# Autodesk Inventor assembly: Top Plate Assembly
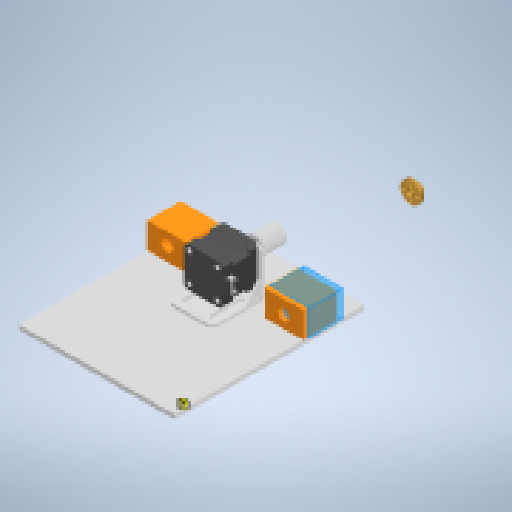
[picture p0: Inventor's stored thumbnail of the model, 512x512]
Saved by Autodesk Inventor 2023.1 (Build 271208000, 208)
## iProperties
Created: 2023-01-31
Part Number: Top Plate Assembly
Document SubType Name: Assembly
Designer: dmargari
Author: dmargari
## iProperties of the stored document Part9.ipt
Created: 2023-02-01
Part Number: Part9
Material: Generic
Document SubType Name: Modeling
Designer: dmargari
Density: 1 g/cm^3
Appearance: Default
Author: dmargari
## iProperties of the stored document JST 2.0 PH - 6 Pin v5.iam
Created: 2023-02-01
Part Number: JST 2.0 PH - 6 Pin
Document SubType Name: Assembly
Designer: dmargari
Author: dmargari
## iProperties of the stored document Shaft.ipt
Created: 2023-02-01
Part Number: Shaft
Material: Steel
Document SubType Name: Modeling
Designer: dmargari
Density: 7.85 g/cm^3
Appearance: Default
Author: dmargari
## iProperties of the stored document M3 x 15mm.iam
Created: 2023-02-01
Part Number: M3 x 15mm
Document SubType Name: Assembly
Designer: dmargari
Author: dmargari
## iProperties of the stored document Pin.ipt
Created: 2023-02-01
Part Number: Pin
Material: Gold
Document SubType Name: Modeling
Designer: dmargari
Density: 19.3 g/cm^3
Appearance: Default
Author: dmargari
## iProperties of the stored document Part13.ipt
Created: 2023-02-01
Part Number: Part13
Material: Generic
Document SubType Name: Modeling
Designer: dmargari
Density: 1 g/cm^3
Appearance: Default
Author: dmargari
## iProperties of the stored document Part11.ipt
Created: 2023-02-01
Part Number: Part11
Material: Generic
Document SubType Name: Modeling
Designer: dmargari
Density: 1 g/cm^3
Appearance: Default
Author: dmargari
## iProperties of the stored document Nema 17 40mm.iam
Created: 2020-03-04
Part Number: Nema 17 40mm
Document SubType Name: Assembly
Designer: dmargari
Sending System: Autodesk Translation Framework v8.12.0.6
Preprocessor: ST-DEVELOPER v18
Title: /Users/nikolajthranecarlsen/Library/Mobile Documents/com~apple~CloudDocs/3D programmer/Rulle gardin/Nema 17 40mm.step
## iProperties of the stored document Mid.ipt
Created: 2023-02-01
Part Number: Mid
Material: Steel
Document SubType Name: Modeling
Designer: dmargari
Density: 7.85 g/cm^3
Appearance: Default
Author: dmargari
## Documents named in this file (14)
- \\icnas3.cc.ic.ac.uk\dmargari\Inventor\Autosampler V3\Top Plate Assembly.iam
- \\icnas3.cc.ic.ac.uk\dmargari\Inventor\Autosampler V3\Top Plate.ipt
- **\\icnas3.cc.ic.ac.uk\dmargari\Inventor\Autosampler V3\Top Plate Assembly.iam*LocalDocs*xAaaaqgbaAaaaaaaaAaaaasfj3f*Nema 17 40mm.iam
- \\icnas3.cc.ic.ac.uk\dmargari\Inventor\Autosampler V3\3rd-party-models\ACME Brass Nut.ipt
- \\icnas3.cc.ic.ac.uk\dmargari\Inventor\Autosampler V3\3rd-party-models\Shaft Coupler 5mm 8mm.ipt
- **\\icnas3.cc.ic.ac.uk\dmargari\Inventor\Autosampler V3\Top Plate Assembly.iam*LocalDocs*xAaaaaubaAaaaaaaaAaaaaqnuYd*Part9.ipt
- **\\icnas3.cc.ic.ac.uk\dmargari\Inventor\Autosampler V3\Top Plate Assembly.iam*LocalDocs*xAaaaalbaAaaaaaaaAaaaq2mvYc*JST 2.0 PH - 6 Pin v5.iam
- **\\icnas3.cc.ic.ac.uk\dmargari\Inventor\Autosampler V3\Top Plate Assembly.iam*LocalDocs*xAaaaqgbaAaaaaaaaAaaaapjfHh*Pin.ipt
- **\\icnas3.cc.ic.ac.uk\dmargari\Inventor\Autosampler V3\Top Plate Assembly.iam*LocalDocs*xAaaaaadaAaaaaaaaAaaaaewrSc*Shaft.ipt
- **\\icnas3.cc.ic.ac.uk\dmargari\Inventor\Autosampler V3\Top Plate Assembly.iam*LocalDocs*xAaaaardaAaaaaaaaAaaaqucmUa*M3 x 15mm.iam
- **\\icnas3.cc.ic.ac.uk\dmargari\Inventor\Autosampler V3\Top Plate Assembly.iam*LocalDocs*xAaaaqtdaAaaaaaaaAaaaah3lHa*Part11.ipt
- **\\icnas3.cc.ic.ac.uk\dmargari\Inventor\Autosampler V3\Top Plate Assembly.iam*LocalDocs*xAaaaaxbaAaaaaaaaAaaaafqyVf*Part13.ipt
- **\\icnas3.cc.ic.ac.uk\dmargari\Inventor\Autosampler V3\Top Plate Assembly.iam*LocalDocs*xAaaaqvaaAaaaaaaaAaaaqrcrCh*Mid.ipt
- \\icnas3.cc.ic.ac.uk\dmargari\Inventor\Autosampler V3\3rd-party-models\nema-17-stepper-motor-24.snapshot.23\Nema 17 40mm.step
## Components (4 placed, 4 different names)
1. Top Plate:1
2. Nema 17 40mm:1 [sub-assembly] — Rigid:2
3. ACME Brass Nut:1
4. Shaft Coupler 5mm 8mm:1 — Rigid:2
## Relationships (1: WeldJoint 1)
- Rigid:2 [WeldJoint] (12 mm): Nema 17 40mm:1 ↔ Shaft Coupler 5mm 8mm:1
